# Autodesk Inventor assembly: shaft_conn
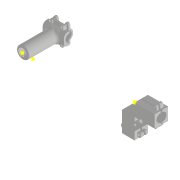
[picture p0: Inventor's stored thumbnail of the model, 180x180]
Saved by Autodesk Inventor 2022 (Build 260153000, 153)
## iProperties
Created: 2022-11-20
Part Number: shaft_conn
Document SubType Name: Assembly
Designer: MVeszpremi
Author: MVeszpremi
## Documents named in this file (4)
- C:\Users\veszp\Dropbox\180DAB CAD\TrayHolder\shaft_conn.iam
- C:\Users\veszp\Dropbox\180DAB CAD\TrayHolder\Shaft_conn_Tensioner.ipt
- C:\Users\veszp\Dropbox\180DAB CAD\TrayHolder\Shaft_Connector_Top.ipt
- C:\Users\veszp\Dropbox\180DAB CAD\TrayHolder\Shaft_Connector_Top_Corner.ipt
## Components (4 placed, 3 different names)
1. Shaft_conn_Tensioner:1 — Mate:1, Mate:2
2. Shaft_Connector_Top:1 — Mate:1, Mate:2
3. Shaft_Connector_Top_Corner:1 — Mate:3, Mate:4
4. Shaft_Connector_Top_Corner:2 — Mate:3, Mate:4
## Relationships (4: Mate 4)
- Mate:1: Shaft_conn_Tensioner:1 ↔ Shaft_Connector_Top:1
- Mate:2: Shaft_conn_Tensioner:1 ↔ Shaft_Connector_Top:1
- Mate:3: Shaft_Connector_Top_Corner:1 ↔ Shaft_Connector_Top_Corner:2
- Mate:4: Shaft_Connector_Top_Corner:1 ↔ Shaft_Connector_Top_Corner:2
